# Autodesk Inventor assembly: RAI Full Assembly
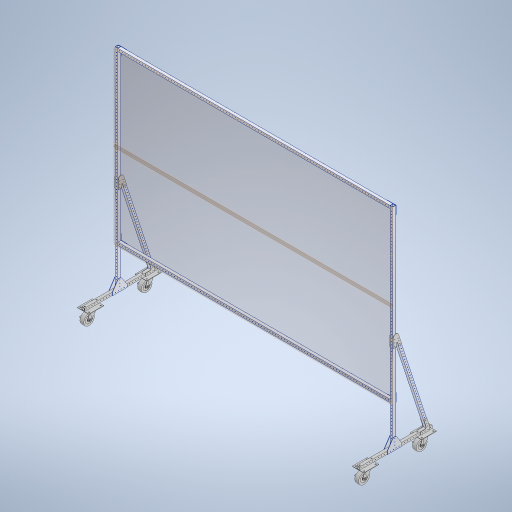
[picture p0: Inventor's stored thumbnail of the model, 512x512]
Saved by Autodesk Inventor 2024 (Build 280153000, 153)
## iProperties
Created: 2023-04-16
Part Number: RAI Full Assembly
Document SubType Name: Assembly
Designer: legom
Author: legom
## Documents named in this file (11)
- C:\Users\legom\Documents\CAD\RAI\RAI Full Assembly.iam
- C:\Users\legom\Documents\CAD\RAI\96 tube.ipt
- C:\Users\legom\Documents\CAD\RAI\Polycarb.ipt
- C:\Users\legom\Documents\CAD\RAI\Short tube.ipt
- C:\Users\legom\Documents\CAD\RAI\Leg_tube.ipt
- C:\Users\legom\Documents\CAD\RAI\T-Gusset.ipt
- C:\Users\legom\Documents\CAD\RAI\L_gusset.ipt
- C:\Users\legom\Documents\CAD\RAI\Angled_bar.ipt
- C:\Users\legom\Documents\CAD\RAI\Bot_ang_gus.ipt
- C:\Users\legom\Documents\CAD\RAI\Top_angled_gusset.ipt
- C:\Users\legom\Documents\CAD\RAI\2407T42_Cart-Smart Caster.ipt
## Components (30 placed, 10 different names)
1. 96 tube:1 — Insert:15, Insert:16, Insert:18
2. Short tube:1 — Insert:2, Insert:3, Insert:13, Insert:14, Insert:19, Insert:20, Insert:21, Insert:22, Insert:27, Insert:30
3. Short tube:2 — Insert:7, Insert:8, Insert:9, Insert:11, Insert:12, Insert:17, Insert:35, Insert:36, Insert:37, Insert:38, Insert:45, Insert:46, Insert:47, Insert:48
4. Polycarb:2 — Insert:9, Insert:10
5. 96 tube:2 — Insert:1, Insert:4, Insert:5, Insert:6, Insert:10
6. Leg_tube:1 — Insert:33, Insert:34, Insert:51, Insert:52, Insert:53, Insert:54
7. Leg_tube:2 — Insert:49, Insert:50, Insert:55, Insert:56, Insert:57, Insert:58
8. L_gusset:1 — Insert:5, Insert:6, Insert:7, Insert:8
9. L_gusset:2 — Insert:1, Insert:2, Insert:3, Insert:4
10. L_gusset:3 — Insert:13, Insert:14, Insert:15, Insert:16
11. L_gusset:4 — Insert:17, Insert:18
12. Angled_bar:1 — Insert:39, Insert:40, Insert:41, Insert:42, Insert:43, Insert:44
13. Angled_bar:2 — Insert:23, Insert:24, Insert:25, Insert:26, Insert:28, Insert:29, Insert:31, Insert:32
14. Bot_ang_gus:2 — Insert:41, Insert:42
15. Bot_ang_gus:1 — Insert:28, Insert:29
16. T-Gusset:1 — Insert:19, Insert:20, Insert:33, Insert:34
17. T-Gusset:2 — Insert:45, Insert:46, Insert:49, Insert:50
18. Top_angled_gusset:1 — Insert:35, Insert:36
19. Top_angled_gusset:2 — Insert:23, Insert:24, Insert:27, Insert:30
20. Polycarb:3 — Insert:11, Insert:12
21. T-Gusset:3 — Insert:21, Insert:22
22. Top_angled_gusset:3 — Insert:25, Insert:26
23. Bot_ang_gus:3 — Insert:31, Insert:32
24. Top_angled_gusset:4 — Insert:37, Insert:38, Insert:39, Insert:40
25. Bot_ang_gus:4 — Insert:43, Insert:44
26. T-Gusset:4 — Insert:47, Insert:48
27. 2407T42_Cart-Smart Caster:1 — Insert:53, Insert:54
28. 2407T42_Cart-Smart Caster:2 — Insert:51, Insert:52
29. 2407T42_Cart-Smart Caster:3 — Insert:55, Insert:56
30. 2407T42_Cart-Smart Caster:4 — Insert:57, Insert:58
## Relationships (58: Insert 58)
- Insert:1: 96 tube:2 ↔ L_gusset:2
- Insert:2: Short tube:1 ↔ L_gusset:2
- Insert:3: Short tube:1 ↔ L_gusset:2
- Insert:4: 96 tube:2 ↔ L_gusset:2
- Insert:5: 96 tube:2 ↔ L_gusset:1
- Insert:6: 96 tube:2 ↔ L_gusset:1
- Insert:7: Short tube:2 ↔ L_gusset:1
- Insert:8: Short tube:2 ↔ L_gusset:1
- Insert:9: Short tube:2 ↔ Polycarb:2
- Insert:10: Polycarb:2 ↔ 96 tube:2
- Insert:11: Short tube:2 ↔ Polycarb:3
- Insert:12: Short tube:2 ↔ Polycarb:3
- Insert:13: Short tube:1 ↔ L_gusset:3
- Insert:14: Short tube:1 ↔ L_gusset:3
- Insert:15: 96 tube:1 ↔ L_gusset:3
- Insert:16: 96 tube:1 ↔ L_gusset:3
- Insert:17: Short tube:2 ↔ L_gusset:4
- Insert:18: 96 tube:1 ↔ L_gusset:4
- Insert:19: Short tube:1 ↔ T-Gusset:1
- Insert:20: Short tube:1 ↔ T-Gusset:1
- Insert:21: Short tube:1 ↔ T-Gusset:3
- Insert:22: Short tube:1 ↔ T-Gusset:3
- Insert:23: Angled_bar:2 ↔ Top_angled_gusset:2
- Insert:24: Angled_bar:2 ↔ Top_angled_gusset:2
- Insert:25: Angled_bar:2 ↔ Top_angled_gusset:3
- Insert:26: Angled_bar:2 ↔ Top_angled_gusset:3
- Insert:27: Short tube:1 ↔ Top_angled_gusset:2
- Insert:28: Angled_bar:2 ↔ Bot_ang_gus:1
- Insert:29: Angled_bar:2 ↔ Bot_ang_gus:1
- Insert:30: Short tube:1 ↔ Top_angled_gusset:2
- Insert:31: Angled_bar:2 ↔ Bot_ang_gus:3
- Insert:32: Angled_bar:2 ↔ Bot_ang_gus:3
- Insert:33: Leg_tube:1 ↔ T-Gusset:1
- Insert:34: Leg_tube:1 ↔ T-Gusset:1
- Insert:35: Short tube:2 ↔ Top_angled_gusset:1
- Insert:36: Short tube:2 ↔ Top_angled_gusset:1
- Insert:37: Short tube:2 ↔ Top_angled_gusset:4
- Insert:38: Short tube:2 ↔ Top_angled_gusset:4
- Insert:39: Angled_bar:1 ↔ Top_angled_gusset:4
- Insert:40: Angled_bar:1 ↔ Top_angled_gusset:4
- Insert:41: Angled_bar:1 ↔ Bot_ang_gus:2
- Insert:42: Angled_bar:1 ↔ Bot_ang_gus:2
- Insert:43: Angled_bar:1 ↔ Bot_ang_gus:4
- Insert:44: Angled_bar:1 ↔ Bot_ang_gus:4
- Insert:45: Short tube:2 ↔ T-Gusset:2
- Insert:46: Short tube:2 ↔ T-Gusset:2
- Insert:47: Short tube:2 ↔ T-Gusset:4
- Insert:48: Short tube:2 ↔ T-Gusset:4
- Insert:49: Leg_tube:2 ↔ T-Gusset:2
- Insert:50: Leg_tube:2 ↔ T-Gusset:2
- Insert:51: Leg_tube:1 ↔ 2407T42_Cart-Smart Caster:2
- Insert:52: Leg_tube:1 ↔ 2407T42_Cart-Smart Caster:2
- Insert:53: Leg_tube:1 ↔ 2407T42_Cart-Smart Caster:1
- Insert:54: Leg_tube:1 ↔ 2407T42_Cart-Smart Caster:1
- Insert:55: Leg_tube:2 ↔ 2407T42_Cart-Smart Caster:3
- Insert:56: Leg_tube:2 ↔ 2407T42_Cart-Smart Caster:3
- Insert:57: Leg_tube:2 ↔ 2407T42_Cart-Smart Caster:4
- Insert:58: Leg_tube:2 ↔ 2407T42_Cart-Smart Caster:4
